# Autodesk Inventor assembly: złożenie gąsienicy
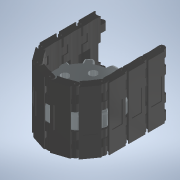
[picture p0: Inventor's stored thumbnail of the model, 180x180]
Saved by Autodesk Inventor 2021 (Build 250183000, 183)
## iProperties
Created: 2021-06-19
Part Number: złożenie gąsienicy
Document SubType Name: Assembly
Designer: Łukasz
Author: Łukasz
## Documents named in this file (3)
- E:\GITHUB_Czołg\Szybki-Czolg-antyRadziecki\złożenie gąsienicy.iam
- E:\GITHUB_Czołg\Szybki-Czolg-antyRadziecki\gąsienica.ipt
- E:\GITHUB_Czołg\Szybki-Czolg-antyRadziecki\koło napędowe.ipt
## Components (11 placed, 2 different names)
1. gąsienica:1 — Rotational:1, Angle:1, Rotational:6, Angle:6
2. gąsienica:2 — Rotational:1, Angle:1, Rotational:2, Angle:2
3. gąsienica:3 — Rotational:5, Angle:5, Rotational:7, Angle:8
4. gąsienica:4 — Rotational:3, Angle:3, Rotational:4, Angle:4, Flush:2
5. gąsienica:5 — Rotational:2, Angle:2, Rotational:3, Angle:3, Mate:1, Flush:1
6. gąsienica:6 — Rotational:6, Angle:6, Rotational:9, Angle:7
7. gąsienica:7 — Rotational:4, Angle:4, Rotational:5, Angle:5
8. gąsienica:8 — Rotational:7, Rotational:8, Angle:8, Angle:9
9. gąsienica:9 — Rotational:8, Angle:9
10. gąsienica:10 — Rotational:9, Angle:7
11. koło napędowe:1 — Mate:1, Flush:1, Flush:2
## Relationships (21: RevoluteJoint 9, Angle 9, Flush 2, Mate 1)
- Rotational:1 [RevoluteJoint]: gąsienica:1 ↔ gąsienica:2
- Angle:1 (-36 deg): gąsienica:1 ↔ gąsienica:2
- Rotational:2 [RevoluteJoint]: gąsienica:2 ↔ gąsienica:5
- Angle:2 (36 deg): gąsienica:2 ↔ gąsienica:5
- Rotational:3 [RevoluteJoint]: gąsienica:4 ↔ gąsienica:5
- Angle:3 (36 deg): gąsienica:4 ↔ gąsienica:5
- Rotational:4 [RevoluteJoint]: gąsienica:4 ↔ gąsienica:7
- Angle:4 (36 deg): gąsienica:4 ↔ gąsienica:7
- Rotational:5 [RevoluteJoint]: gąsienica:3 ↔ gąsienica:7
- Angle:5 (36 deg): gąsienica:3 ↔ gąsienica:7
- Rotational:6 [RevoluteJoint]: gąsienica:1 ↔ gąsienica:6
- Angle:6 (0 deg): gąsienica:1 ↔ gąsienica:6
- Rotational:7 [RevoluteJoint]: gąsienica:3 ↔ gąsienica:8
- Rotational:8 [RevoluteJoint]: gąsienica:8 ↔ gąsienica:9
- Rotational:9 [RevoluteJoint]: gąsienica:6 ↔ gąsienica:10
- Angle:7 (0 deg): gąsienica:6 ↔ gąsienica:10
- Angle:8 (0 deg): gąsienica:3 ↔ gąsienica:8
- Angle:9 (0 deg): gąsienica:8 ↔ gąsienica:9
- Mate:1 (1 mm): gąsienica:5 ↔ koło napędowe:1
- Flush:1: gąsienica:5 ↔ koło napędowe:1
- Flush:2: gąsienica:4 ↔ koło napędowe:1
